# Autodesk Inventor assembly: Outer_Tube_Adjst_Asm_Test
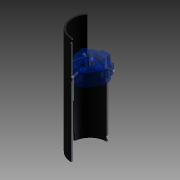
[picture p0: Inventor's stored thumbnail of the model, 180x180]
Saved by Autodesk Inventor 2011 SP2 (Build 150309200, 309)
## iProperties
Created: 2012-05-23
Part Number: Outer_Tube_Adjst_Asm_Test
Document SubType Name: Assembly
Designer: sungwook
Author: sungwook
## Documents named in this file (4)
- C:\Users\sungwook\Documents\Inventor\Micron20_Base_Tube_Adjst\Outer_Tube_Adjst_Asm_Test.iam
- C:\Users\sungwook\Documents\Inventor\Micron20_Base_Tube_Adjst\Outer_Tube.ipt
- C:\Users\sungwook\Documents\Inventor\Micron20_Base_Tube_Adjst\Parts\Main\Platform_Base_20mm_Rev2.ipt
- C:\Users\sungwook\Documents\Inventor\Content Center Files\R2011\en-US\ANSI B18.6.3(00)\ANSI B18.6.3 - 0-80 UNF - 0.1875(32).ipt
## Components (5 placed, 3 different names)
1. Outer_Tube:1 — Mate:1, Mate:3, Mate:5
2. Platform_Base_20mm_Rev2:1 — Mate:1, Mate:2, Mate:3, Mate:4, Mate:5
3. Cross Recessed 100° Flat Countersunk Head Machine Screw - Type I - Inch 0-80 UNF x 0.1875:1 — Mate:4
4. Cross Recessed 100° Flat Countersunk Head Machine Screw - Type I - Inch 0-80 UNF x 0.1875:2
5. Cross Recessed 100° Flat Countersunk Head Machine Screw - Type I - Inch 0-80 UNF x 0.1875:3
## Component patterns: (3 elements, first: Cross Recessed 100° Flat Countersunk Head Machine Screw - Type I - Inch 0-80 UNF x 0.1875:1)
## Relationships (5: Mate 5)
- Mate:1: Outer_Tube:1 ↔ Platform_Base_20mm_Rev2:1
- Mate:2: Platform_Base_20mm_Rev2:1
- Mate:3: Outer_Tube:1 ↔ Platform_Base_20mm_Rev2:1
- Mate:5: Outer_Tube:1 ↔ Platform_Base_20mm_Rev2:1
- Mate:4: Platform_Base_20mm_Rev2:1 ↔ Cross Recessed 100° Flat Countersunk Head Machine Screw - Type I - Inch 0-80 UNF x 0.1875:1
